# Autodesk Inventor assembly: FlyWheel_Assembly_Jan21
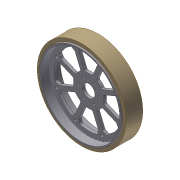
[picture p0: Inventor's stored thumbnail of the model, 180x180]
Saved by Autodesk Inventor 2012 (Build 160160000, 160)
## iProperties
Created: 2012-01-22
Part Number: FlyWheel_Assembly_Jan21
Document SubType Name: Assembly
Designer: JesseK
Mass: 1912.31 g
Surface Area: 2592.68 cm^2
Volume: 753.287 cm^3
Density: 2.53862 g/cm^3
Author: JesseK
## Documents named in this file (7)
- Z:\UserData\Documents\Inventor\team1885frc\Robot2012\Shooter\FlyWheel_Assembly_Jan21.iam
- Z:\UserData\Documents\Inventor\team1885frc\Robot2012\Shooter\FlyWheel_Base_Jan21.ipt
- Z:\UserData\Documents\Inventor\team1885frc\Robot2012\Shooter\FlyWheel_Weight_Jan21.ipt
- Z:\UserData\Documents\Inventor\team1885frc\Robot2012\Shooter\FlyWheel_TreadMount_Jan21.ipt
- Z:\UserData\Documents\Inventor\Content Center Files\R2012\en-US\ANSI B18.6.3(54)\ANSI B18.6.3 - 1_4 - 20 x 2(8).ipt
- Z:\UserData\Documents\Inventor\team1885frc\Robot2012\Shooter\FlyWheel_Tread.ipt
- Z:\UserData\Documents\Inventor\team1885frc\Hardware\Nuts\LockNut_0.375_24.ipt
## Components (27 placed, 6 different names)
1. FlyWheel_Base_Jan21:1 — Mate:3, Mate:4, Mate:5, Mate:9, Mate:10, Mate:11, Mate:14, Mate:15, Mate:17, Mate:19, Mate:22, Mate:23, Mate:25, Flush:1, Mate:59, Mate:60, Mate:61, Mate:62, Mate:63, Mate:64, Mate:65, Mate:66, Mate:67, Mate:68, Mate:69, Mate:70
2. FlyWheel_Weight_Jan21:3 — Mate:15, Mate:17, Mate:23, Mate:49, Mate:50
3. FlyWheel_Weight_Jan21:5 — Mate:14, Mate:19, Mate:22, Mate:45, Mate:46
4. FlyWheel_Weight_Jan21:7 — Mate:9, Mate:10, Mate:11, Mate:28, Mate:29, Mate:36, Mate:37
5. FlyWheel_Weight_Jan21:8 — Mate:3, Mate:4, Mate:5, Mate:32, Mate:33, Mate:40, Mate:41
6. FlyWheel_TreadMount_Jan21:1 — Mate:25, Flush:1, Mate:42, Flush:2
7. Slotted Pan Head Machine Screw - Inch 1/4 - 20 x 2:1 — Mate:56
8. Slotted Pan Head Machine Screw - Inch 1/4 - 20 x 2:2 — Mate:55
9. Slotted Pan Head Machine Screw - Inch 1/4 - 20 x 2:3 — Mate:28, Mate:36, Mate:57
10. Slotted Pan Head Machine Screw - Inch 1/4 - 20 x 2:4 — Mate:29, Mate:37, Mate:58
11. Slotted Pan Head Machine Screw - Inch 1/4 - 20 x 2:5 — Mate:54
12. Slotted Pan Head Machine Screw - Inch 1/4 - 20 x 2:6 — Mate:53
13. Slotted Pan Head Machine Screw - Inch 1/4 - 20 x 2:7 — Mate:32, Mate:41, Mate:51
14. Slotted Pan Head Machine Screw - Inch 1/4 - 20 x 2:8 — Mate:33, Mate:40, Mate:52
15. FlyWheel_Tread:1 — Mate:42, Flush:2
16. LockNut_0.375_24:1 — Mate:50, Mate:51
17. LockNut_0.375_24:2 — Mate:49, Mate:52
18. LockNut_0.375_24:3 — Mate:53
19. LockNut_0.375_24:4 — Mate:54
20. LockNut_0.375_24:5 — Mate:46, Mate:58
21. LockNut_0.375_24:6 — Mate:45, Mate:57
22. LockNut_0.375_24:7 — Mate:56
23. LockNut_0.375_24:8 — Mate:55
24. FlyWheel_Weight_Jan21:9 — Mate:59, Mate:61, Mate:62
25. FlyWheel_Weight_Jan21:10 — Mate:65, Mate:67, Mate:68
26. FlyWheel_Weight_Jan21:11 — Mate:66, Mate:69, Mate:70
27. FlyWheel_Weight_Jan21:12 — Mate:60, Mate:63, Mate:64
## Relationships (48: Mate 46, Flush 2)
- Mate:3: FlyWheel_Base_Jan21:1 ↔ FlyWheel_Weight_Jan21:8
- Mate:4: FlyWheel_Base_Jan21:1 ↔ FlyWheel_Weight_Jan21:8
- Mate:5: FlyWheel_Base_Jan21:1 ↔ FlyWheel_Weight_Jan21:8
- Mate:9: FlyWheel_Base_Jan21:1 ↔ FlyWheel_Weight_Jan21:7
- Mate:10: FlyWheel_Base_Jan21:1 ↔ FlyWheel_Weight_Jan21:7
- Mate:11: FlyWheel_Base_Jan21:1 ↔ FlyWheel_Weight_Jan21:7
- Mate:14: FlyWheel_Base_Jan21:1 ↔ FlyWheel_Weight_Jan21:5
- Mate:15: FlyWheel_Base_Jan21:1 ↔ FlyWheel_Weight_Jan21:3
- Mate:17: FlyWheel_Base_Jan21:1 ↔ FlyWheel_Weight_Jan21:3
- Mate:19: FlyWheel_Base_Jan21:1 ↔ FlyWheel_Weight_Jan21:5
- Mate:22: FlyWheel_Base_Jan21:1 ↔ FlyWheel_Weight_Jan21:5
- Mate:23: FlyWheel_Base_Jan21:1 ↔ FlyWheel_Weight_Jan21:3
- Mate:25: FlyWheel_Base_Jan21:1 ↔ FlyWheel_TreadMount_Jan21:1
- Flush:1 (-19.05 mm): FlyWheel_Base_Jan21:1 ↔ FlyWheel_TreadMount_Jan21:1
- Mate:28: FlyWheel_Weight_Jan21:7 ↔ Slotted Pan Head Machine Screw - Inch 1/4 - 20 x 2:3
- Mate:29: FlyWheel_Weight_Jan21:7 ↔ Slotted Pan Head Machine Screw - Inch 1/4 - 20 x 2:4
- Mate:32: FlyWheel_Weight_Jan21:8 ↔ Slotted Pan Head Machine Screw - Inch 1/4 - 20 x 2:7
- Mate:33: FlyWheel_Weight_Jan21:8 ↔ Slotted Pan Head Machine Screw - Inch 1/4 - 20 x 2:8
- Mate:36: FlyWheel_Weight_Jan21:7 ↔ Slotted Pan Head Machine Screw - Inch 1/4 - 20 x 2:3
- Mate:37: FlyWheel_Weight_Jan21:7 ↔ Slotted Pan Head Machine Screw - Inch 1/4 - 20 x 2:4
- Mate:40: FlyWheel_Weight_Jan21:8 ↔ Slotted Pan Head Machine Screw - Inch 1/4 - 20 x 2:8
- Mate:41: FlyWheel_Weight_Jan21:8 ↔ Slotted Pan Head Machine Screw - Inch 1/4 - 20 x 2:7
- Mate:42: FlyWheel_TreadMount_Jan21:1 ↔ FlyWheel_Tread:1
- Flush:2 (3.175 mm): FlyWheel_TreadMount_Jan21:1 ↔ FlyWheel_Tread:1
- Mate:45: FlyWheel_Weight_Jan21:5 ↔ LockNut_0.375_24:6
- Mate:46: FlyWheel_Weight_Jan21:5 ↔ LockNut_0.375_24:5
- Mate:49: FlyWheel_Weight_Jan21:3 ↔ LockNut_0.375_24:2
- Mate:50: FlyWheel_Weight_Jan21:3 ↔ LockNut_0.375_24:1
- Mate:51: Slotted Pan Head Machine Screw - Inch 1/4 - 20 x 2:7 ↔ LockNut_0.375_24:1
- Mate:52: Slotted Pan Head Machine Screw - Inch 1/4 - 20 x 2:8 ↔ LockNut_0.375_24:2
- Mate:53: Slotted Pan Head Machine Screw - Inch 1/4 - 20 x 2:6 ↔ LockNut_0.375_24:3
- Mate:54: Slotted Pan Head Machine Screw - Inch 1/4 - 20 x 2:5 ↔ LockNut_0.375_24:4
- Mate:55: Slotted Pan Head Machine Screw - Inch 1/4 - 20 x 2:2 ↔ LockNut_0.375_24:8
- Mate:56: Slotted Pan Head Machine Screw - Inch 1/4 - 20 x 2:1 ↔ LockNut_0.375_24:7
- Mate:57: Slotted Pan Head Machine Screw - Inch 1/4 - 20 x 2:3 ↔ LockNut_0.375_24:6
- Mate:58: Slotted Pan Head Machine Screw - Inch 1/4 - 20 x 2:4 ↔ LockNut_0.375_24:5
- Mate:59: FlyWheel_Base_Jan21:1 ↔ FlyWheel_Weight_Jan21:9
- Mate:60: FlyWheel_Base_Jan21:1 ↔ FlyWheel_Weight_Jan21:12
- Mate:61: FlyWheel_Base_Jan21:1 ↔ FlyWheel_Weight_Jan21:9
- Mate:62: FlyWheel_Base_Jan21:1 ↔ FlyWheel_Weight_Jan21:9
- Mate:63: FlyWheel_Base_Jan21:1 ↔ FlyWheel_Weight_Jan21:12
- Mate:64: FlyWheel_Base_Jan21:1 ↔ FlyWheel_Weight_Jan21:12
- Mate:65: FlyWheel_Base_Jan21:1 ↔ FlyWheel_Weight_Jan21:10
- Mate:66: FlyWheel_Base_Jan21:1 ↔ FlyWheel_Weight_Jan21:11
- Mate:67: FlyWheel_Base_Jan21:1 ↔ FlyWheel_Weight_Jan21:10
- Mate:68: FlyWheel_Base_Jan21:1 ↔ FlyWheel_Weight_Jan21:10
- Mate:69: FlyWheel_Base_Jan21:1 ↔ FlyWheel_Weight_Jan21:11
- Mate:70: FlyWheel_Base_Jan21:1 ↔ FlyWheel_Weight_Jan21:11
